# Autodesk Inventor assembly: samling
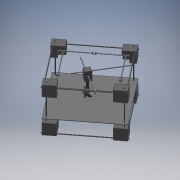
[picture p0: Inventor's stored thumbnail of the model, 180x180]
Saved by Autodesk Inventor 2018 (Build 220112000, 112)
## iProperties
Created: 2018-01-24
Part Number: samling
Document SubType Name: Assembly
Designer: MikkelS
Author: MikkelS
## Documents named in this file (18)
- C:\Users\MikkelS\Documents\Inventor\Teknikproj2\samling.iam
- C:\Users\MikkelS\Documents\Inventor\Teknikproj2\AIS2016\16N2A12A010 -(0N).iam
- C:\Users\MikkelS\Documents\Inventor\Teknikproj2\[ZPT08UNK6-04-A8]-[AIS2016]\AIS2016\ZPT08UNK6-04-A8_N.iam
- C:\Users\MikkelS\Documents\Inventor\Teknikproj2\Centerhoved.ipt
- C:\Users\MikkelS\Documents\Inventor\Teknikproj2\pin.ipt
- C:\Users\MikkelS\Documents\Inventor\Teknikproj2\69141997-9-ball_bearing_lm6uu\ball_bearing_lm6uu.ipt
- C:\Users\MikkelS\Documents\Inventor\Teknikproj2\Tophjørne1.ipt
- C:\Users\MikkelS\Documents\Inventor\Teknikproj2\gevindstang.ipt
- C:\Users\MikkelS\Documents\Inventor\Teknikproj2\69146584-9-roulement_626-2rsh_2\roulement_626-2rsh_2.iam
- C:\Users\MikkelS\Documents\Inventor\Teknikproj2\løbestang.ipt
- C:\Users\MikkelS\Documents\Inventor\Teknikproj2\Tophjørnemirror.ipt
- C:\Users\MikkelS\Documents\Inventor\Teknikproj2\løbestang1.ipt
- C:\Users\MikkelS\Documents\Inventor\Teknikproj2\gevindstang1.ipt
- C:\Users\MikkelS\Documents\Inventor\Teknikproj2\Bundhjørne1.ipt
- C:\Users\MikkelS\Documents\Inventor\Teknikproj2\Bundhjørnemirror.ipt
- C:\Users\MikkelS\Documents\Inventor\Teknikproj2\løbestangcenter.ipt
- C:\Users\MikkelS\Documents\Inventor\Teknikproj2\bundplade.ipt
- C:\Users\MikkelS\Documents\Inventor\Teknikproj2\gevindstang300.ipt
## Components (45 placed, 17 different names)
1. 16N2A12A010 -(0N):1 [sub-assembly] — Mate:1, Mate:2, Mate:3, Mate:4, Mate:5
2. ZPT08UNK6-04-A8_N:1 [sub-assembly] — Mate:1, Mate:2
3. Centerhoved:1 — Mate:3, Mate:4, Flush:1, Mate:6, Mate:7, Flush:2, Flush:3, Flush:25
4. pin:1 — Mate:5, Flush:1
5. ball_bearing_lm6uu:1 — Mate:6, Flush:3, Mate:83
6. ball_bearing_lm6uu:2 — Mate:7, Flush:2, Mate:82
7. Tophjørne1:1 — Mate:14, Flush:11, Mate:15, Flush:12, Flush:15, Flush:26, Flush:27, Flush:28, Flush:29, Mate:52, Mate:63, Flush:33, Mate:69, Mate:92, Flush:45
8. Tophjørne1:3 — Mate:16, Flush:13, Flush:15, Mate:43, Mate:44, Flush:27, Flush:30, Mate:65, Mate:67, Flush:35, Mate:88, Flush:43
9. roulement_626-2rsh_2:1 [sub-assembly] — Mate:14, Flush:11, Mate:22
10. roulement_626-2rsh_2:2 [sub-assembly] — Mate:16, Flush:13, Mate:59
11. roulement_626-2rsh_2:3 [sub-assembly] — Mate:15, Flush:12, Mate:62
12. løbestang:3 — Mate:22, Mate:46, Mate:51, Mate:52, Mate:84
13. Tophjørnemirror:1 — Flush:25, Mate:35, Mate:36, Mate:37, Mate:38, Flush:26, Flush:29, Flush:30, Mate:55, Flush:32, Flush:34, Mate:90, Flush:44
14. Tophjørnemirror:2 — Mate:39, Mate:40, Mate:41, Mate:42, Flush:28, Mate:51, Mate:64, Mate:66, Mate:68, Mate:91, Flush:46
15. roulement_626-2rsh_2:4 [sub-assembly] — Mate:43, Mate:44, Mate:49
16. roulement_626-2rsh_2:5 [sub-assembly] — Mate:37, Mate:38, Mate:61
17. roulement_626-2rsh_2:6 [sub-assembly] — Mate:40, Mate:41, Mate:60
18. roulement_626-2rsh_2:7 [sub-assembly] — Mate:35, Mate:36, Mate:48
19. roulement_626-2rsh_2:8 [sub-assembly] — Mate:39, Mate:42, Mate:46
20. løbestang:5 — Mate:48, Mate:49, Mate:55, Mate:86
21. løbestang1:1 — Mate:59, Mate:60, Mate:64, Mate:65, Mate:85
22. løbestang1:2 — Mate:61, Mate:62, Mate:63, Mate:87
23. gevindstang:12 — Mate:66, Flush:33
24. gevindstang:13 — Mate:67, Flush:32
25. gevindstang1:1 — Mate:68, Flush:35
26. gevindstang1:2 — Mate:69, Flush:34
27. Bundhjørne1:1 — Mate:72, Flush:36, Mate:80, Mate:93
28. Bundhjørnemirror:1 — Mate:73, Mate:75, Mate:95
29. gevindstang:14 — Mate:72, Mate:73, Flush:36
30. Bundhjørne1:2 — Mate:76, Flush:37, Mate:78, Flush:41, Mate:94
31. gevindstang1:3 — Mate:75, Mate:76, Flush:37
32. Bundhjørnemirror:2 — Mate:79, Flush:38, Mate:81, Flush:39, Flush:42, Mate:89, Flush:47
33. gevindstang:15 — Mate:78, Mate:79, Flush:38
34. gevindstang1:4 — Mate:80, Mate:81, Flush:39
35. løbestangcenter:1 — Mate:82
36. løbestangcenter:2 — Mate:83
37. ball_bearing_lm6uu:3 — Mate:86
38. ball_bearing_lm6uu:4 — Mate:87
39. ball_bearing_lm6uu:5 — Mate:85
40. ball_bearing_lm6uu:6 — Mate:84
41. bundplade:1 — Flush:41, Flush:42
42. gevindstang300:1 — Mate:90, Flush:44, Mate:94
43. gevindstang300:2 — Mate:91, Flush:46, Mate:93
44. gevindstang300:3 — Mate:88, Flush:43, Mate:89, Flush:47
45. gevindstang300:4 — Mate:92, Flush:45, Mate:95
## Relationships (88: Mate 60, Flush 28)
- Mate:1: 16N2A12A010 -(0N):1 ↔ ZPT08UNK6-04-A8_N:1
- Mate:2: 16N2A12A010 -(0N):1 ↔ ZPT08UNK6-04-A8_N:1
- Mate:3: 16N2A12A010 -(0N):1 ↔ Centerhoved:1
- Mate:4: 16N2A12A010 -(0N):1 ↔ Centerhoved:1
- Mate:5: 16N2A12A010 -(0N):1 ↔ pin:1
- Flush:1: Centerhoved:1 ↔ pin:1
- Mate:6: Centerhoved:1 ↔ ball_bearing_lm6uu:1
- Mate:7: Centerhoved:1 ↔ ball_bearing_lm6uu:2
- Flush:2 (8.5 mm): Centerhoved:1 ↔ ball_bearing_lm6uu:2
- Flush:3 (8.5 mm): Centerhoved:1 ↔ ball_bearing_lm6uu:1
- Mate:14: Tophjørne1:1 ↔ roulement_626-2rsh_2:1
- Flush:11: Tophjørne1:1 ↔ roulement_626-2rsh_2:1
- Mate:15: Tophjørne1:1 ↔ roulement_626-2rsh_2:3
- Flush:12: Tophjørne1:1 ↔ roulement_626-2rsh_2:3
- Mate:16: Tophjørne1:3 ↔ roulement_626-2rsh_2:2
- Flush:13: Tophjørne1:3 ↔ roulement_626-2rsh_2:2
- Mate:22: roulement_626-2rsh_2:1 ↔ løbestang:3
- Flush:15: Tophjørne1:1 ↔ Tophjørne1:3
- Flush:25: Centerhoved:1 ↔ Tophjørnemirror:1
- Mate:35: Tophjørnemirror:1 ↔ roulement_626-2rsh_2:7
- Mate:36: Tophjørnemirror:1 ↔ roulement_626-2rsh_2:7
- Mate:37: Tophjørnemirror:1 ↔ roulement_626-2rsh_2:5
- Mate:38: Tophjørnemirror:1 ↔ roulement_626-2rsh_2:5
- Mate:39: Tophjørnemirror:2 ↔ roulement_626-2rsh_2:8
- Mate:40: Tophjørnemirror:2 ↔ roulement_626-2rsh_2:6
- Mate:41: Tophjørnemirror:2 ↔ roulement_626-2rsh_2:6
- Mate:42: Tophjørnemirror:2 ↔ roulement_626-2rsh_2:8
- Mate:43: Tophjørne1:3 ↔ roulement_626-2rsh_2:4
- Mate:44: Tophjørne1:3 ↔ roulement_626-2rsh_2:4
- Mate:46: løbestang:3 ↔ roulement_626-2rsh_2:8
- Flush:26: Tophjørne1:1 ↔ Tophjørnemirror:1
- Flush:27: Tophjørne1:1 ↔ Tophjørne1:3
- Flush:28: Tophjørne1:1 ↔ Tophjørnemirror:2
- Flush:29: Tophjørne1:1 ↔ Tophjørnemirror:1
- Mate:48: roulement_626-2rsh_2:7 ↔ løbestang:5
- Flush:30: Tophjørne1:3 ↔ Tophjørnemirror:1
- Mate:49: roulement_626-2rsh_2:4 ↔ løbestang:5
- Mate:51: løbestang:3 ↔ Tophjørnemirror:2
- Mate:52: Tophjørne1:1 ↔ løbestang:3
- Mate:55: Tophjørnemirror:1 ↔ løbestang:5
- Mate:59: roulement_626-2rsh_2:2 ↔ løbestang1:1
- Mate:60: roulement_626-2rsh_2:6 ↔ løbestang1:1
- Mate:61: roulement_626-2rsh_2:5 ↔ løbestang1:2
- Mate:62: roulement_626-2rsh_2:3 ↔ løbestang1:2
- Mate:63: Tophjørne1:1 ↔ løbestang1:2
- Mate:64: Tophjørnemirror:2 ↔ løbestang1:1
- Mate:65: Tophjørne1:3 ↔ løbestang1:1
- Mate:66: Tophjørnemirror:2 ↔ gevindstang:12
- Mate:67: Tophjørne1:3 ↔ gevindstang:13
- Flush:32 (-5 mm): Tophjørnemirror:1 ↔ gevindstang:13
- Flush:33 (-5 mm): Tophjørne1:1 ↔ gevindstang:12
- Mate:68: Tophjørnemirror:2 ↔ gevindstang1:1
- Mate:69: Tophjørne1:1 ↔ gevindstang1:2
- Flush:34 (-5 mm): Tophjørnemirror:1 ↔ gevindstang1:2
- Flush:35 (-5 mm): Tophjørne1:3 ↔ gevindstang1:1
- Mate:72: Bundhjørne1:1 ↔ gevindstang:14
- Mate:73: Bundhjørnemirror:1 ↔ gevindstang:14
- Flush:36 (-5 mm): Bundhjørne1:1 ↔ gevindstang:14
- Mate:75: Bundhjørnemirror:1 ↔ gevindstang1:3
- Mate:76: Bundhjørne1:2 ↔ gevindstang1:3
- Flush:37 (-5 mm): Bundhjørne1:2 ↔ gevindstang1:3
- Mate:78: Bundhjørne1:2 ↔ gevindstang:15
- Mate:79: Bundhjørnemirror:2 ↔ gevindstang:15
- Flush:38 (-5 mm): Bundhjørnemirror:2 ↔ gevindstang:15
- Mate:80: Bundhjørne1:1 ↔ gevindstang1:4
- Mate:81: Bundhjørnemirror:2 ↔ gevindstang1:4
- Flush:39 (-5 mm): Bundhjørnemirror:2 ↔ gevindstang1:4
- Mate:82: ball_bearing_lm6uu:2 ↔ løbestangcenter:1
- Mate:83: ball_bearing_lm6uu:1 ↔ løbestangcenter:2
- Mate:84: løbestang:3 ↔ ball_bearing_lm6uu:6
- Mate:85: løbestang1:1 ↔ ball_bearing_lm6uu:5
- Mate:86: løbestang:5 ↔ ball_bearing_lm6uu:3
- Mate:87: løbestang1:2 ↔ ball_bearing_lm6uu:4
- Flush:41: Bundhjørne1:2 ↔ bundplade:1
- Flush:42: Bundhjørnemirror:2 ↔ bundplade:1
- Mate:88: Tophjørne1:3 ↔ gevindstang300:3
- Flush:43 (-5 mm): Tophjørne1:3 ↔ gevindstang300:3
- Mate:89: Bundhjørnemirror:2 ↔ gevindstang300:3
- Mate:90: Tophjørnemirror:1 ↔ gevindstang300:1
- Flush:44 (-5 mm): Tophjørnemirror:1 ↔ gevindstang300:1
- Mate:91: Tophjørnemirror:2 ↔ gevindstang300:2
- Mate:92: Tophjørne1:1 ↔ gevindstang300:4
- Flush:45 (-5 mm): Tophjørne1:1 ↔ gevindstang300:4
- Flush:46 (-5 mm): Tophjørnemirror:2 ↔ gevindstang300:2
- Mate:93: Bundhjørne1:1 ↔ gevindstang300:2
- Mate:94: Bundhjørne1:2 ↔ gevindstang300:1
- Mate:95: Bundhjørnemirror:1 ↔ gevindstang300:4
- Flush:47 (-5 mm): Bundhjørnemirror:2 ↔ gevindstang300:3
